# Autodesk Inventor assembly: リンク_ふくらはぎ_後ろ_1
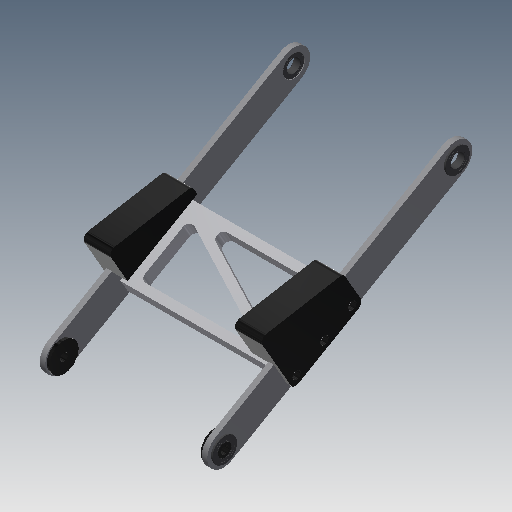
[picture p0: Inventor's stored thumbnail of the model, 512x512]
Saved by Autodesk Inventor 2017.3 (Build 213256000, 256)
## iProperties
Created: 2016-04-29
Part Number: リンク_ふくらはぎ_後ろ_1
Document SubType Name: Assembly
Designer: hiroaki
Mass: 54.0583 g
Surface Area: 163.215 cm^2
Volume: 16.5096 cm^3
Density: 3.27436 g/cm^3
Author: hiroaki
## Documents named in this file (7)
- C:\Users\haya\Desktop\GankenKun0_5\下半身\リンク\ふくらはぎ\リンク_ふくらはぎ_後ろ_1.iam
- C:\Users\haya\Desktop\GankenKun0_5\下半身\リンク\ふくらはぎ\リンク_ふくらはぎ_メインフレーム_1_2.ipt
- C:\Users\haya\Desktop\GankenKun0_5\既製品\NSK_RB_MF85ZZ\MF85ZZ.iam
- C:\Users\haya\Desktop\GankenKun0_5\下半身\リンク\スペーサ\足首_スペーサ_1_1.ipt
- C:\Users\haya\Desktop\GankenKun0_5\下半身\リンク\ふくらはぎ\リンク_ふくらはぎ_サブフレーム_1_5.ipt
- C:\Users\haya\Desktop\GankenKun0_5\下半身\リンク\ふくらはぎ\リンク_ふくらはぎ_サブフレーム_1_5_MIR.ipt
- C:\Users\haya\Desktop\GankenKun0_5\下半身\リンク\ふくらはぎ\リンク_ふくらはぎ_サブフレーム_1_2(予備案).ipt
## Components (11 placed, 6 different names)
1. リンク_ふくらはぎ_メインフレーム_1_2:1 — 挿入:7, 挿入:8, 挿入:11, 挿入:28, 挿入:29, 挿入:30, 挿入:34, 挿入:35, 挿入:36
2. リンク_ふくらはぎ_メインフレーム_1_2:2 — 挿入:9, 挿入:10, 挿入:12, 挿入:31, 挿入:32, 挿入:33, 挿入:37, 挿入:38, 挿入:39
3. MF85ZZ:1 [sub-assembly] — 挿入:7
4. MF85ZZ:2 [sub-assembly] — 挿入:8
5. MF85ZZ:3 [sub-assembly] — 挿入:9
6. MF85ZZ:4 [sub-assembly] — 挿入:10
7. 足首_スペーサ_1_1:1 — 挿入:12
8. 足首_スペーサ_1_1:2 — 挿入:11
9. リンク_ふくらはぎ_サブフレーム_1_5:1 — 挿入:28, 挿入:29, 挿入:30
10. リンク_ふくらはぎ_サブフレーム_1_5_MIR:1 — 挿入:31, 挿入:32, 挿入:33
11. リンク_ふくらはぎ_サブフレーム_1_2(予備案):1 — 挿入:34, 挿入:35, 挿入:36, 挿入:37, 挿入:38, 挿入:39
## Relationships (18: Insert 18)
- 挿入:7 [Insert]: リンク_ふくらはぎ_メインフレーム_1_2:1 ↔ MF85ZZ:1
- 挿入:8 [Insert]: リンク_ふくらはぎ_メインフレーム_1_2:1 ↔ MF85ZZ:2
- 挿入:9 [Insert]: リンク_ふくらはぎ_メインフレーム_1_2:2 ↔ MF85ZZ:3
- 挿入:10 [Insert]: リンク_ふくらはぎ_メインフレーム_1_2:2 ↔ MF85ZZ:4
- 挿入:11 [Insert]: リンク_ふくらはぎ_メインフレーム_1_2:1 ↔ 足首_スペーサ_1_1:2
- 挿入:12 [Insert]: リンク_ふくらはぎ_メインフレーム_1_2:2 ↔ 足首_スペーサ_1_1:1
- 挿入:28 [Insert]: リンク_ふくらはぎ_メインフレーム_1_2:1 ↔ リンク_ふくらはぎ_サブフレーム_1_5:1
- 挿入:29 [Insert]: リンク_ふくらはぎ_メインフレーム_1_2:1 ↔ リンク_ふくらはぎ_サブフレーム_1_5:1
- 挿入:30 [Insert]: リンク_ふくらはぎ_メインフレーム_1_2:1 ↔ リンク_ふくらはぎ_サブフレーム_1_5:1
- 挿入:31 [Insert]: リンク_ふくらはぎ_メインフレーム_1_2:2 ↔ リンク_ふくらはぎ_サブフレーム_1_5_MIR:1
- 挿入:32 [Insert]: リンク_ふくらはぎ_メインフレーム_1_2:2 ↔ リンク_ふくらはぎ_サブフレーム_1_5_MIR:1
- 挿入:33 [Insert]: リンク_ふくらはぎ_メインフレーム_1_2:2 ↔ リンク_ふくらはぎ_サブフレーム_1_5_MIR:1
- 挿入:34 [Insert]: リンク_ふくらはぎ_メインフレーム_1_2:1 ↔ リンク_ふくらはぎ_サブフレーム_1_2(予備案):1
- 挿入:35 [Insert]: リンク_ふくらはぎ_メインフレーム_1_2:1 ↔ リンク_ふくらはぎ_サブフレーム_1_2(予備案):1
- 挿入:36 [Insert]: リンク_ふくらはぎ_メインフレーム_1_2:1 ↔ リンク_ふくらはぎ_サブフレーム_1_2(予備案):1
- 挿入:37 [Insert]: リンク_ふくらはぎ_メインフレーム_1_2:2 ↔ リンク_ふくらはぎ_サブフレーム_1_2(予備案):1
- 挿入:38 [Insert]: リンク_ふくらはぎ_メインフレーム_1_2:2 ↔ リンク_ふくらはぎ_サブフレーム_1_2(予備案):1
- 挿入:39 [Insert]: リンク_ふくらはぎ_メインフレーム_1_2:2 ↔ リンク_ふくらはぎ_サブフレーム_1_2(予備案):1
